# Autodesk Inventor assembly: Strap mount
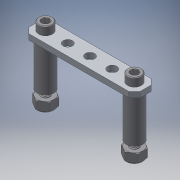
[picture p0: Inventor's stored thumbnail of the model, 180x180]
Saved by Autodesk Inventor 2018 (Build 220112000, 112)
## iProperties
Created: 2020-01-28
Part Number: Strap mount
Document SubType Name: Assembly
Designer: maste
Author: maste
## Documents named in this file (5)
- C:\Users\maste\OneDrive\Documents\GitHub\2020CAD\Drivebase AM14U1\Part Files\Strap mount.iam
- C:\Users\maste\OneDrive\Documents\GitHub\2020CAD\Drivebase AM14U1\Part Files\Bolts\92196A277_18-8 STAINLESS STEEL SOCKET HEAD CAP SCREW.ipt
- C:\Users\maste\OneDrive\Documents\GitHub\2020CAD\Drivebase AM14U1\Part Files\Locknuts\91831A411_TYPE 18-8 STAINLESS STL NYLON-INSERT LOCKNUT.ipt
- C:\Users\maste\OneDrive\Documents\GitHub\2020CAD\Drivebase AM14U1\Part Files\battery strap spacer.ipt
- C:\Users\maste\OneDrive\Documents\GitHub\2020CAD\Drivebase AM14U1\Part Files\am-3960 AM14U4 Vertical Battery Mount Strap Clamp.ipt
## Components (7 placed, 4 different names)
1. 92196A277_18-8 STAINLESS STEEL SOCKET HEAD CAP SCREW:1 — Mate:2, Mate:4, Mate:6, Mate:10, Rotation:4
2. 92196A277_18-8 STAINLESS STEEL SOCKET HEAD CAP SCREW:2 — Mate:1, Mate:3, Mate:5, Mate:9, Rotation:1
3. 91831A411_TYPE 18-8 STAINLESS STL NYLON-INSERT LOCKNUT:1 — Mate:10, Mate:11, Rotation:4, Rotation:5
4. 91831A411_TYPE 18-8 STAINLESS STL NYLON-INSERT LOCKNUT:2 — Mate:9, Mate:12, Rotation:1, Rotation:2
5. battery strap spacer:1 — Mate:6, Mate:7, Mate:11, Rotation:5, Rotation:6
6. battery strap spacer:2 — Mate:5, Mate:8, Mate:12, Rotation:2, Rotation:3
7. am-3960 AM14U4 Vertical Battery Mount Strap Clamp:1 — Mate:1, Mate:2, Mate:3, Mate:4, Mate:7, Mate:8, Rotation:3, Rotation:6
## Relationships (18: Mate 12, RelateRotation 6)
- Mate:1: 92196A277_18-8 STAINLESS STEEL SOCKET HEAD CAP SCREW:2 ↔ am-3960 AM14U4 Vertical Battery Mount Strap Clamp:1
- Mate:2: 92196A277_18-8 STAINLESS STEEL SOCKET HEAD CAP SCREW:1 ↔ am-3960 AM14U4 Vertical Battery Mount Strap Clamp:1
- Mate:3: 92196A277_18-8 STAINLESS STEEL SOCKET HEAD CAP SCREW:2 ↔ am-3960 AM14U4 Vertical Battery Mount Strap Clamp:1
- Mate:4: 92196A277_18-8 STAINLESS STEEL SOCKET HEAD CAP SCREW:1 ↔ am-3960 AM14U4 Vertical Battery Mount Strap Clamp:1
- Mate:5: 92196A277_18-8 STAINLESS STEEL SOCKET HEAD CAP SCREW:2 ↔ battery strap spacer:2
- Mate:6: 92196A277_18-8 STAINLESS STEEL SOCKET HEAD CAP SCREW:1 ↔ battery strap spacer:1
- Mate:7: battery strap spacer:1 ↔ am-3960 AM14U4 Vertical Battery Mount Strap Clamp:1
- Mate:8: battery strap spacer:2 ↔ am-3960 AM14U4 Vertical Battery Mount Strap Clamp:1
- Mate:9: 92196A277_18-8 STAINLESS STEEL SOCKET HEAD CAP SCREW:2 ↔ 91831A411_TYPE 18-8 STAINLESS STL NYLON-INSERT LOCKNUT:2
- Mate:10: 92196A277_18-8 STAINLESS STEEL SOCKET HEAD CAP SCREW:1 ↔ 91831A411_TYPE 18-8 STAINLESS STL NYLON-INSERT LOCKNUT:1
- Mate:11 (3.175 mm): 91831A411_TYPE 18-8 STAINLESS STL NYLON-INSERT LOCKNUT:1 ↔ battery strap spacer:1
- Mate:12 (3.175 mm): 91831A411_TYPE 18-8 STAINLESS STL NYLON-INSERT LOCKNUT:2 ↔ battery strap spacer:2
- Rotation:1 [RelateRotation] (1 ul): 92196A277_18-8 STAINLESS STEEL SOCKET HEAD CAP SCREW:2 ↔ 91831A411_TYPE 18-8 STAINLESS STL NYLON-INSERT LOCKNUT:2
- Rotation:2 [RelateRotation] (1 ul): 91831A411_TYPE 18-8 STAINLESS STL NYLON-INSERT LOCKNUT:2 ↔ battery strap spacer:2
- Rotation:3 [RelateRotation] (1 ul): battery strap spacer:2 ↔ am-3960 AM14U4 Vertical Battery Mount Strap Clamp:1
- Rotation:4 [RelateRotation] (1 ul): 92196A277_18-8 STAINLESS STEEL SOCKET HEAD CAP SCREW:1 ↔ 91831A411_TYPE 18-8 STAINLESS STL NYLON-INSERT LOCKNUT:1
- Rotation:5 [RelateRotation] (1 ul): 91831A411_TYPE 18-8 STAINLESS STL NYLON-INSERT LOCKNUT:1 ↔ battery strap spacer:1
- Rotation:6 [RelateRotation] (1 ul): battery strap spacer:1 ↔ am-3960 AM14U4 Vertical Battery Mount Strap Clamp:1
